# Autodesk Inventor assembly: AXb3
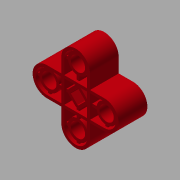
[picture p0: Inventor's stored thumbnail of the model, 180x180]
Saved by Autodesk Inventor 2019.3 (Build 233278000, 278)
## iProperties
Created: 2019-02-07
Part Number: AXb3
Document SubType Name: Assembly
Designer: Varga Daniel
Author: Varga Daniel
## Documents named in this file (5)
- C:\!_Dani\!_cloud\OneDrive\!_munka\Revolution\RevvyDemoKit\Structural parts\Beams\Axle Beams\AXbX.iam
- C:\!_Dani\!_cloud\OneDrive\!_munka\Revolution\RevvyDemoKit\Structural parts\Beams\beam_single_end_part.ipt
- C:\!_Dani\!_cloud\OneDrive\!_munka\Revolution\RevvyDemoKit\Structural parts\Beams\Axle Beams\Axle beam base.ipt
- AXb1.iam
- AXb3.iam
## Components (5 placed, 2 different names)
1. beam_single_end_part:1 — Flush:1, Flush:2, Mate:1
2. beam_single_end_part:2 — Mate:2, Flush:3, Flush:4
3. beam_single_end_part:3 — Mate:3, Flush:5, Flush:6
4. beam_single_end_part:4 — Flush:7, Flush:8, Mate:4
5. Axle beam base:2 — Flush:1, Flush:2, Mate:1, Mate:2, Flush:3, Flush:4, Mate:3, Flush:5, Flush:6, Flush:7, Flush:8, Mate:4
## Relationships (12: Flush 8, Mate 4)
- Flush:1: beam_single_end_part:1 ↔ Axle beam base:2
- Flush:2: beam_single_end_part:1 ↔ Axle beam base:2
- Mate:1: beam_single_end_part:1 ↔ Axle beam base:2
- Mate:2: beam_single_end_part:2 ↔ Axle beam base:2
- Flush:3: beam_single_end_part:2 ↔ Axle beam base:2
- Flush:4: beam_single_end_part:2 ↔ Axle beam base:2
- Mate:3: beam_single_end_part:3 ↔ Axle beam base:2
- Flush:5: beam_single_end_part:3 ↔ Axle beam base:2
- Flush:6: beam_single_end_part:3 ↔ Axle beam base:2
- Flush:7: beam_single_end_part:4 ↔ Axle beam base:2
- Flush:8: beam_single_end_part:4 ↔ Axle beam base:2
- Mate:4: beam_single_end_part:4 ↔ Axle beam base:2
